# Autodesk Inventor assembly: BD_test
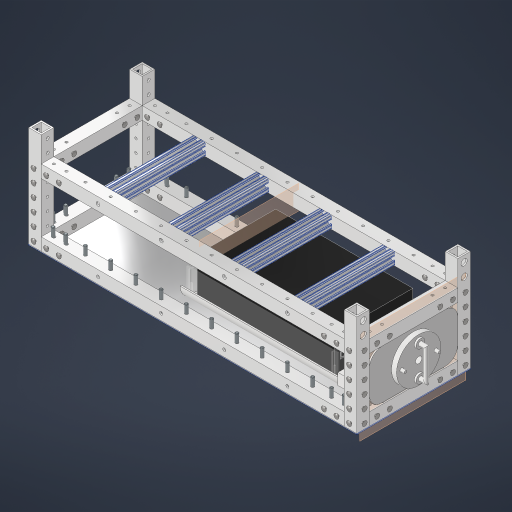
[picture p0: Inventor's stored thumbnail of the model, 512x512]
Saved by Autodesk Inventor 2024 (Build 280153000, 153)
## iProperties
Created: 2024-01-25
Part Number: BD_test
Document SubType Name: Assembly
Designer: seene
Author: seene
## Documents named in this file (4)
- C:\Users\calvi\OneDrive\Robocup Rescue\Chassis\Battery Drawer\BD_test.iam
- C:\Users\calvi\OneDrive\Robocup Rescue\Chassis\Frame\Centerpiece with DTconnector.iam
- Centerpiece.iam
- C:\Users\calvi\OneDrive\Robocup Rescue\Chassis\Battery Drawer\Sheet_Assembly.iam
## Components (2 placed, 2 different names)
1. Centerpiece:1 [sub-assembly] — Slider:1, Flush:3
2. Sheet_Assembly:1 [sub-assembly] — Slider:1, Flush:3
## Relationships (2: TranslationJoint 1, Flush 1)
- Slider:1 [TranslationJoint]: Centerpiece:1 ↔ Sheet_Assembly:1
- Flush:3: Centerpiece:1 ↔ Sheet_Assembly:1
